# Autodesk Inventor assembly: Upper Arm
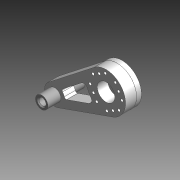
[picture p0: Inventor's stored thumbnail of the model, 180x180]
Saved by Autodesk Inventor 2014 SP1 (Build 180222100, 222)
## iProperties
Created: 2013-12-25
Part Number: Upper Arm
Document SubType Name: Assembly
Designer: tom
Author: tom
## Documents named in this file (4)
- C:\Users\tom\Documents\GitHub\Delta_Robots\Delatabot - Small Model\Imported Components\Deltabot - Small Model\Upper Arm.iam
- C:\Users\tom\Documents\GitHub\Delta_Robots\Delatabot - Small Model\Imported Components\Deltabot - Small Model\Component6.ipt
- C:\Users\tom\Documents\GitHub\Delta_Robots\Delatabot - Small Model\Imported Components\Deltabot - Small Model\Component7.ipt
- C:\Users\tom\Documents\GitHub\Delta_Robots\Delatabot - Small Model\Imported Components\Deltabot - Small Model\Linkage Mount.ipt
## Components (3 placed, 3 different names)
1. Servo Hub 1
2. Linkage Mount:1 — Mate:4, Flush:1
3. Servo Arm 1 — Mate:4, Flush:1
## Relationships (5: Mate 4, Flush 1)
- [Mate]: Servo Hub 1 ↔ Servo Arm 1
- [Mate]: Servo Hub 1 ↔ Servo Arm 1
- [Mate]: Servo Hub 1 ↔ Servo Arm 1
- Mate:4: Linkage Mount:1 ↔ Servo Arm 1
- Flush:1 (-6.67 mm): Linkage Mount:1 ↔ Servo Arm 1
